# Autodesk Inventor assembly: 胴体_1
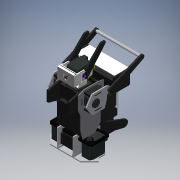
[picture p0: Inventor's stored thumbnail of the model, 180x180]
Saved by Autodesk Inventor 2018 (Build 220112000, 112)
## iProperties
Created: 2016-05-03
Part Number: 胴体_1
Document SubType Name: Assembly
Designer: hiroaki
Mass: 1526.48 g
Surface Area: 4615.97 cm^2
Volume: 792.505 cm^3
Density: 1.92615 g/cm^3
Author: hiroaki
## Documents named in this file (21)
- Z:\OPR\OpenPlatform_ver1_0\上半身\胴体\胴体_1.iam
- Z:\OPR\OpenPlatform_ver1_0\既製品\B3M11xx.ipt
- Z:\OPR\OpenPlatform_ver1_0\既製品\B3M10xx.ipt
- Z:\OPR\OpenPlatform_ver1_0\上半身\胴体\胴体_メインフレーム_1_1.ipt
- Z:\OPR\OpenPlatform_ver1_0\上半身\胴体\胴体_メインフレーム_1_2.ipt
- Z:\OPR\OpenPlatform_ver1_0\上半身\胴体\胴体_サブフレーム_1_1.ipt
- Z:\OPR\OpenPlatform_ver1_0\上半身\胴体\胴体_サブフレーム_1_2.ipt
- Z:\OPR\OpenPlatform_ver1_0\上半身\胴体\胴体_サブフレーム_1_3.ipt
- Z:\OPR\OpenPlatform_ver1_0\上半身\胴体\胴体_サブフレーム_1_4.ipt
- Z:\OPR\OpenPlatform_ver1_0\上半身\頭\頭_1.iam
- Z:\OPR\OpenPlatform_ver1_0\上半身\頭\頭_1_2.iam
- Z:\OPR\OpenPlatform_ver1_0\上半身\胴体\胴体_サブフレーム_1_6.ipt
- Z:\OPR\OpenPlatform_ver1_0\上半身\胴体\胴体_サブフレーム_1_6_MIR.ipt
- Z:\OPR\OpenPlatform_ver1_0\上半身\胴体\胴体_サブフレーム_1_1_MIR.ipt
- Z:\OPR\OpenPlatform_ver1_0\上半身\胴体\胴体_サブフレーム_1_7.ipt
- Z:\OPR\OpenPlatform_ver1_0\上半身\胴体\胴体_サブフレーム_1_7_MIR.ipt
- Z:\OPR\OpenPlatform_ver1_0\上半身\胴体\胴体_メインフレーム_1_12.ipt
- Z:\OPR\OpenPlatform_ver1_0\上半身\胴体\胴体_メインフレーム_1_13.ipt
- Z:\OPR\OpenPlatform_ver1_0\上半身\コックピット\コックピット_2\コックピット_2.iam
- Z:\OPR\OpenPlatform_ver1_0\上半身\胴体\胴体_サブフレーム_1_12.ipt
- Z:\OPR\OpenPlatform_ver1_0\既製品\AETTF8-135-M3-N3.ipt
## Components (31 placed, 19 different names)
1. 胴体_メインフレーム_1_1:1 — 挿入:1, 挿入:2, 挿入:3, 挿入:4, 挿入:5, 挿入:6, 挿入:43, 挿入:44, 挿入:120, 挿入:121
2. 胴体_メインフレーム_1_2:1 — 挿入:23, 挿入:24, 挿入:25, 挿入:28
3. 胴体_メインフレーム_1_12:1 — 挿入:148, 挿入:149, 挿入:150, 挿入:151
4. 胴体_サブフレーム_1_1:1 — 挿入:43, 挿入:44, 挿入:118, 挿入:119
5. 胴体_サブフレーム_1_2:1 — フラッシュ:1, メイト:4
6. 胴体_サブフレーム_1_3:1 — 挿入:150, 挿入:151, 挿入:162, 挿入:163, 挿入:168, 挿入:169, 挿入:192, 挿入:193, メイト:4, 挿入:231, 挿入:232, 挿入:238
7. 胴体_サブフレーム_1_4:1 — 挿入:57, 挿入:58, 挿入:148, 挿入:149, 挿入:152, 挿入:153
8. 胴体_サブフレーム_1_6:1 — 挿入:118, 挿入:119
9. 胴体_サブフレーム_1_7:1 — 挿入:231, 挿入:232
10. 胴体_サブフレーム_1_12:1 — 挿入:247
11. 胴体_メインフレーム_1_13:1 — 挿入:190, 挿入:191, 挿入:192, 挿入:193
12. B3M11xx:5 — 挿入:104, 角度:21
13. B3M11xx:4 — 挿入:57, 挿入:58
14. B3M11xx:3 — 角度:1, 挿入:76, 挿入:77
15. B3M11xx:2 — 挿入:2, 挿入:4, 挿入:5, 挿入:23, 挿入:25
16. B3M11xx:1 — 角度:1, 挿入:1, 挿入:3, 挿入:6, 挿入:24, 挿入:28
17. 頭_1_2:1 [sub-assembly] — 挿入:105, 角度:22
18. 頭_1:1 [sub-assembly] — 挿入:104, 挿入:105, 角度:21, 角度:22
19. コックピット_2:1 [sub-assembly] — 挿入:237, 挿入:238
20. AETTF8-135-M3-N3:1 — 挿入:246, 挿入:247
21. 胴体_サブフレーム_1_12:2 — 挿入:246
22. 胴体_メインフレーム_1_13:2 — 挿入:168, 挿入:169, 挿入:170, 挿入:171
23. 胴体_メインフレーム_1_12:2 — 挿入:152, 挿入:153, 挿入:162, 挿入:163
24. 胴体_メインフレーム_1_12:3 — 挿入:154, 挿入:155, 挿入:156, 挿入:157
25. 胴体_メインフレーム_1_12:4 — 挿入:158, 挿入:159, 挿入:160, 挿入:161
26. 胴体_サブフレーム_1_7_MIR:1 — 挿入:233, 挿入:234
27. 胴体_サブフレーム_1_6_MIR:1 — 挿入:122, 挿入:123
28. 胴体_サブフレーム_1_1_MIR:1 — 挿入:120, 挿入:121, 挿入:122, 挿入:123, メイト:7
29. 胴体_サブフレーム_1_2:2 — フラッシュ:1, メイト:5, メイト:7
30. 胴体_サブフレーム_1_3:2 — 挿入:156, 挿入:157, 挿入:160, 挿入:161, 挿入:170, 挿入:171, 挿入:190, 挿入:191, メイト:5, 挿入:233, 挿入:234, 挿入:237
31. 胴体_サブフレーム_1_4:2 — 挿入:76, 挿入:77, 挿入:154, 挿入:155, 挿入:158, 挿入:159
## Relationships (63: Insert 56, Angle 3, Mate 3, Flush 1)
- 角度:1 [Angle] (0 deg): B3M11xx:3 ↔ B3M11xx:1
- 挿入:1 [Insert]: 胴体_メインフレーム_1_1:1 ↔ B3M11xx:1
- 挿入:2 [Insert]: 胴体_メインフレーム_1_1:1 ↔ B3M11xx:2
- 挿入:3 [Insert]: 胴体_メインフレーム_1_1:1 ↔ B3M11xx:1
- 挿入:4 [Insert]: 胴体_メインフレーム_1_1:1 ↔ B3M11xx:2
- 挿入:5 [Insert]: 胴体_メインフレーム_1_1:1 ↔ B3M11xx:2
- 挿入:6 [Insert]: 胴体_メインフレーム_1_1:1 ↔ B3M11xx:1
- 挿入:23 [Insert]: 胴体_メインフレーム_1_2:1 ↔ B3M11xx:2
- 挿入:24 [Insert]: 胴体_メインフレーム_1_2:1 ↔ B3M11xx:1
- 挿入:25 [Insert]: 胴体_メインフレーム_1_2:1 ↔ B3M11xx:2
- 挿入:28 [Insert]: 胴体_メインフレーム_1_2:1 ↔ B3M11xx:1
- 挿入:43 [Insert]: 胴体_メインフレーム_1_1:1 ↔ 胴体_サブフレーム_1_1:1
- 挿入:44 [Insert]: 胴体_メインフレーム_1_1:1 ↔ 胴体_サブフレーム_1_1:1
- 挿入:57 [Insert]: 胴体_サブフレーム_1_4:1 ↔ B3M11xx:4
- 挿入:58 [Insert]: 胴体_サブフレーム_1_4:1 ↔ B3M11xx:4
- 挿入:76 [Insert]: B3M11xx:3 ↔ 胴体_サブフレーム_1_4:2
- 挿入:77 [Insert]: B3M11xx:3 ↔ 胴体_サブフレーム_1_4:2
- 挿入:104 [Insert]: B3M11xx:5 ↔ 頭_1:1
- 挿入:105 [Insert]: 頭_1_2:1 ↔ 頭_1:1
- 角度:21 [Angle] (0 deg): B3M11xx:5 ↔ 頭_1:1
- 角度:22 [Angle] (0 deg): 頭_1_2:1 ↔ 頭_1:1
- 挿入:118 [Insert]: 胴体_サブフレーム_1_1:1 ↔ 胴体_サブフレーム_1_6:1
- 挿入:119 [Insert]: 胴体_サブフレーム_1_1:1 ↔ 胴体_サブフレーム_1_6:1
- 挿入:120 [Insert]: 胴体_メインフレーム_1_1:1 ↔ 胴体_サブフレーム_1_1_MIR:1
- 挿入:121 [Insert]: 胴体_メインフレーム_1_1:1 ↔ 胴体_サブフレーム_1_1_MIR:1
- 挿入:122 [Insert]: 胴体_サブフレーム_1_6_MIR:1 ↔ 胴体_サブフレーム_1_1_MIR:1
- 挿入:123 [Insert]: 胴体_サブフレーム_1_6_MIR:1 ↔ 胴体_サブフレーム_1_1_MIR:1
- 挿入:148 [Insert]: 胴体_メインフレーム_1_12:1 ↔ 胴体_サブフレーム_1_4:1
- 挿入:149 [Insert]: 胴体_メインフレーム_1_12:1 ↔ 胴体_サブフレーム_1_4:1
- 挿入:150 [Insert]: 胴体_メインフレーム_1_12:1 ↔ 胴体_サブフレーム_1_3:1
- 挿入:151 [Insert]: 胴体_メインフレーム_1_12:1 ↔ 胴体_サブフレーム_1_3:1
- 挿入:152 [Insert]: 胴体_サブフレーム_1_4:1 ↔ 胴体_メインフレーム_1_12:2
- 挿入:153 [Insert]: 胴体_サブフレーム_1_4:1 ↔ 胴体_メインフレーム_1_12:2
- 挿入:154 [Insert]: 胴体_メインフレーム_1_12:3 ↔ 胴体_サブフレーム_1_4:2
- 挿入:155 [Insert]: 胴体_メインフレーム_1_12:3 ↔ 胴体_サブフレーム_1_4:2
- 挿入:156 [Insert]: 胴体_メインフレーム_1_12:3 ↔ 胴体_サブフレーム_1_3:2
- 挿入:157 [Insert]: 胴体_メインフレーム_1_12:3 ↔ 胴体_サブフレーム_1_3:2
- 挿入:158 [Insert]: 胴体_メインフレーム_1_12:4 ↔ 胴体_サブフレーム_1_4:2
- 挿入:159 [Insert]: 胴体_メインフレーム_1_12:4 ↔ 胴体_サブフレーム_1_4:2
- 挿入:160 [Insert]: 胴体_メインフレーム_1_12:4 ↔ 胴体_サブフレーム_1_3:2
- 挿入:161 [Insert]: 胴体_メインフレーム_1_12:4 ↔ 胴体_サブフレーム_1_3:2
- 挿入:162 [Insert]: 胴体_サブフレーム_1_3:1 ↔ 胴体_メインフレーム_1_12:2
- 挿入:163 [Insert]: 胴体_サブフレーム_1_3:1 ↔ 胴体_メインフレーム_1_12:2
- 挿入:168 [Insert]: 胴体_サブフレーム_1_3:1 ↔ 胴体_メインフレーム_1_13:2
- 挿入:169 [Insert]: 胴体_サブフレーム_1_3:1 ↔ 胴体_メインフレーム_1_13:2
- 挿入:170 [Insert]: 胴体_メインフレーム_1_13:2 ↔ 胴体_サブフレーム_1_3:2
- 挿入:171 [Insert]: 胴体_メインフレーム_1_13:2 ↔ 胴体_サブフレーム_1_3:2
- 挿入:190 [Insert]: 胴体_メインフレーム_1_13:1 ↔ 胴体_サブフレーム_1_3:2
- 挿入:191 [Insert]: 胴体_メインフレーム_1_13:1 ↔ 胴体_サブフレーム_1_3:2
- 挿入:192 [Insert]: 胴体_サブフレーム_1_3:1 ↔ 胴体_メインフレーム_1_13:1
- 挿入:193 [Insert]: 胴体_サブフレーム_1_3:1 ↔ 胴体_メインフレーム_1_13:1
- フラッシュ:1 [Flush]: 胴体_サブフレーム_1_2:1 ↔ 胴体_サブフレーム_1_2:2
- メイト:4 [Mate]: 胴体_サブフレーム_1_2:1 ↔ 胴体_サブフレーム_1_3:1
- メイト:5 [Mate]: 胴体_サブフレーム_1_2:2 ↔ 胴体_サブフレーム_1_3:2
- メイト:7 [Mate]: 胴体_サブフレーム_1_1_MIR:1 ↔ 胴体_サブフレーム_1_2:2
- 挿入:231 [Insert]: 胴体_サブフレーム_1_3:1 ↔ 胴体_サブフレーム_1_7:1
- 挿入:232 [Insert]: 胴体_サブフレーム_1_3:1 ↔ 胴体_サブフレーム_1_7:1
- 挿入:233 [Insert]: 胴体_サブフレーム_1_7_MIR:1 ↔ 胴体_サブフレーム_1_3:2
- 挿入:234 [Insert]: 胴体_サブフレーム_1_7_MIR:1 ↔ 胴体_サブフレーム_1_3:2
- 挿入:237 [Insert]: コックピット_2:1 ↔ 胴体_サブフレーム_1_3:2
- 挿入:238 [Insert]: 胴体_サブフレーム_1_3:1 ↔ コックピット_2:1
- 挿入:246 [Insert]: AETTF8-135-M3-N3:1 ↔ 胴体_サブフレーム_1_12:2
- 挿入:247 [Insert]: 胴体_サブフレーム_1_12:1 ↔ AETTF8-135-M3-N3:1
